# Autodesk Inventor assembly: NarrowWall
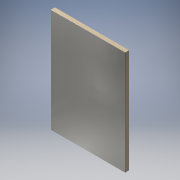
[picture p0: Inventor's stored thumbnail of the model, 180x180]
Saved by Autodesk Inventor 2017 (Build 210142000, 142)
## iProperties
Created: 2016-12-13
Part Number: NarrowWall
Document SubType Name: Assembly
Designer: umr
Author: umr
## Documents named in this file (3)
- D:\SeniorProject\Models2\Case\NarrowWall.iam
- D:\SeniorProject\Models2\Case\InsulatorWallNorrow.ipt
- D:\SeniorProject\Models2\Case\ReflectorWallNorrow.ipt
## Components (2 placed, 2 different names)
1. InsulatorWallNorrow:1 — Mate:1, Flush:1, Flush:2
2. ReflectorWallNorrow:1 — Mate:1, Flush:1, Flush:2
## Relationships (3: Flush 2, Mate 1)
- Mate:1: InsulatorWallNorrow:1 ↔ ReflectorWallNorrow:1
- Flush:1: InsulatorWallNorrow:1 ↔ ReflectorWallNorrow:1
- Flush:2: InsulatorWallNorrow:1 ↔ ReflectorWallNorrow:1
